# Autodesk Inventor assembly: elric20-2A
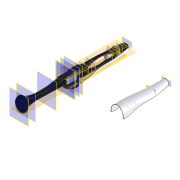
[picture p0: Inventor's stored thumbnail of the model, 180x180]
Saved by Autodesk Inventor 2020.2 (Build 242310000, 310)
## iProperties
Created: 2020-04-12
Part Number: elric20-2A
Document SubType Name: Assembly
Designer: Bardo91
Author: Bardo91
## Documents named in this file (11)
- D:\programming\elric\hardware\2. arm\elric20-02A.iam
- D:\programming\elric\hardware\2. arm\wrist.ipt
- D:\programming\elric\hardware\2. arm\forearm.ipt
- D:\programming\elric\hardware\2. arm\case\arm_case_1.ipt
- D:\programming\elric\hardware\2. arm\case\arm_case_2.ipt
- D:\programming\elric\hardware\2. arm\motor_dc_20d_12v.ipt
- D:\programming\elric\hardware\2. arm\elbow_gear_ext.ipt
- D:\programming\elric\hardware\2. arm\elbow_gear_int_1.ipt
- D:\programming\elric\hardware\2. arm\elbow_gear_int_2.ipt
- D:\programming\elric\hardware\2. arm\arm.ipt
- D:\programming\elric\hardware\2. arm\motor_dc_12v_90d.ipt
## Components (12 placed, 9 different names)
1. wrist:1 — Mate:3, Mate:4
2. forearm:1 — Mate:1, Mate:2, Mate:3, Mate:4, Mate:16, Mate:17, Mate:18, Mate:23, Mate:24, Mate:25, Mate:26, Mate:27, Mate:28
3. motor_dc_20d_12v:1 — Mate:1, Mate:2
4. Spur Gear1:1 — Mate:16, Mate:17, Mate:18, Mate:20
5. Spur Gear2:1
6. Spur Gear2:2
7. Spur Gear2:3
8. Spur Gear2:4 — Mate:15, Mate:22
9. arm:1 — Mate:19, Mate:21
10. motor_dc_12v_90d:1 — Mate:15, Mate:19, Mate:20, Mate:21, Mate:22
11. arm_case_1:1 — Mate:26, Mate:27, Mate:28
12. arm_case_2:1 — Mate:23, Mate:24, Mate:25
## Relationships (26: Mate 22, Flush 4)
- Mate:1: forearm:1 ↔ motor_dc_20d_12v:1
- Mate:2: forearm:1 ↔ motor_dc_20d_12v:1
- Mate:3: wrist:1 ↔ forearm:1
- Mate:4 (0.5 mm): wrist:1 ↔ forearm:1
- [Mate]: Spur Gear2:2 ↔ arm:1
- [Flush]: Spur Gear2:3 ↔ Spur Gear2:4
- [Flush]: Spur Gear2:1 ↔ Spur Gear2:4
- [Flush]: Spur Gear2:2 ↔ Spur Gear2:4
- [Mate]: Spur Gear1:1 ↔ Spur Gear2:4
- [Flush]: Spur Gear1:1 ↔ Spur Gear2:4
- [Mate]: Spur Gear2:1 ↔ arm:1
- [Mate]: Spur Gear2:3 ↔ arm:1
- Mate:15: Spur Gear2:4 ↔ motor_dc_12v_90d:1
- Mate:16: forearm:1 ↔ Spur Gear1:1
- Mate:17: forearm:1 ↔ Spur Gear1:1
- Mate:18: forearm:1 ↔ Spur Gear1:1
- Mate:19: arm:1 ↔ motor_dc_12v_90d:1
- Mate:20: Spur Gear1:1 ↔ motor_dc_12v_90d:1
- Mate:21: arm:1 ↔ motor_dc_12v_90d:1
- Mate:22: Spur Gear2:4 ↔ motor_dc_12v_90d:1
- Mate:23: forearm:1 ↔ arm_case_2:1
- Mate:24: forearm:1 ↔ arm_case_2:1
- Mate:25: forearm:1 ↔ arm_case_2:1
- Mate:26: forearm:1 ↔ arm_case_1:1
- Mate:27: forearm:1 ↔ arm_case_1:1
- Mate:28: forearm:1 ↔ arm_case_1:1
